# Autodesk Inventor assembly: meccanum_wheel_base_norm.0004
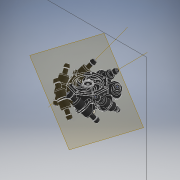
[picture p0: Inventor's stored thumbnail of the model, 180x180]
Saved by Autodesk Inventor 2022 (Build 260153000, 153)
## iProperties
Created: 2023-01-06
Part Number: meccanum_wheel_base_norm.0004
Document SubType Name: Assembly
Designer: Иван Петров
Author: Иван Петров
## Documents named in this file (4)
- C:\Users\Ivan Petrov\Documents\GitHub\OmniBot\design\standart_components\VEX Meccanum wheel\meccanum_wheel_base_norm.0004.iam
- C:\Users\Ivan Petrov\Documents\GitHub\OmniBot\design\standart_components\VEX Meccanum wheel\meccanum_wheel_base.ipt
- C:\Users\Ivan Petrov\Documents\GitHub\OmniBot\design\standart_components\vex_mechanum_adapter.ipt
- C:\Users\Ivan Petrov\Documents\GitHub\OmniBot\design\standart_components\vex_mechanum_adapter (1) зеркальный.ipt
## Components (3 placed, 3 different names)
1. meccanum_wheel_base:1 — Совмещение:1, Совмещение:2, Заподлицо:1, Совмещение:3, Совмещение:4, Совмещение:5, Совмещение:6, Совмещение:7, Совмещение:8, Совмещение:9, Совмещение:10
2. vex_mechanum_adapter (1) зеркальный:1 — Совмещение:5, Совмещение:6, Совмещение:7
3. vex_mechanum_adapter:1 — Совмещение:8, Совмещение:9, Совмещение:10
## Relationships (11: Mate 10, Flush 1)
- Совмещение:1 [Mate]: meccanum_wheel_base:1
- Совмещение:2 [Mate]: meccanum_wheel_base:1
- Заподлицо:1 [Flush] (-1 mm): meccanum_wheel_base:1
- Совмещение:3 [Mate]: meccanum_wheel_base:1
- Совмещение:4 [Mate]: meccanum_wheel_base:1
- Совмещение:5 [Mate]: meccanum_wheel_base:1 ↔ vex_mechanum_adapter (1) зеркальный:1
- Совмещение:6 [Mate]: meccanum_wheel_base:1 ↔ vex_mechanum_adapter (1) зеркальный:1
- Совмещение:7 [Mate]: meccanum_wheel_base:1 ↔ vex_mechanum_adapter (1) зеркальный:1
- Совмещение:8 [Mate]: meccanum_wheel_base:1 ↔ vex_mechanum_adapter:1
- Совмещение:9 [Mate]: meccanum_wheel_base:1 ↔ vex_mechanum_adapter:1
- Совмещение:10 [Mate]: meccanum_wheel_base:1 ↔ vex_mechanum_adapter:1
